# Autodesk Inventor assembly: LegAssemblyRightFront
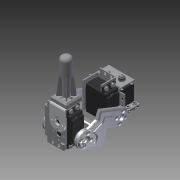
[picture p0: Inventor's stored thumbnail of the model, 180x180]
Saved by Autodesk Inventor 2015 (Build 190159000, 159)
## iProperties
Created: 2015-05-22
Part Number: LegAssemblyRightFront
Document SubType Name: Assembly
Designer: Quinn
Author: Quinn
## Documents named in this file (8)
- C:\Users\Quinn\Desktop\3DCNC Design\InventorModels\Assemblies\LegAssemblyRightFront.iam
- C:\Users\Quinn\Desktop\3DCNC Design\InventorModels\Assemblies\FXR_HipServo.iam
- C:\Users\Quinn\Desktop\3DCNC Design\InventorModels\Assemblies\LegAssemblyRightFront\Design Accelerator\Bolted Connection1.iam
- C:\Users\Quinn\Desktop\3DCNC Design\InventorModels\Assemblies\Knee_RightFront.iam
- C:\Users\Quinn\Desktop\3DCNC Design\InventorModels\Assemblies\FXL_HipServo.iam
- C:\Users\Quinn\Desktop\3DCNC Design\InventorModels\Assemblies\Foot.iam
- C:\Users\Quinn\Desktop\3DCNC Design\InventorModels\Assemblies\LegAssemblyRightFront\Design Accelerator\Bolted Connection2.iam
- C:\Users\Quinn\Desktop\3DCNC Design\InventorModels\Assemblies\LegAssemblyRightFront\Design Accelerator\Bolted Connection3.iam
## Components (8 placed, 5 different names)
1. FXR_HipServo:1 [sub-assembly] — Mate:1, Mate:2, Mate:3
2. FXR_HipServo:2 [sub-assembly] — Mate:1, Rotational:1
3. Bolted Connection:1 [sub-assembly] — Mate:2, Mate:3
4. Knee_RightFront:1 [sub-assembly] — Rotational:1, Rotational:2
5. FXL_HipServo:1 [sub-assembly] — Rotational:2, Mate:4, Mate:5, Mate:6
6. Foot:1 [sub-assembly] — Mate:4, Mate:5, Mate:6, Mate:7, Mate:8, Mate:9, Mate:10
7. Bolted Connection:2 [sub-assembly] — Mate:7, Mate:8
8. Bolted Connection:3 [sub-assembly] — Mate:9, Mate:10
## Relationships (12: Mate 10, RevoluteJoint 2)
- Mate:1: FXR_HipServo:1 ↔ FXR_HipServo:2
- Mate:2: FXR_HipServo:1 ↔ Bolted Connection:1
- Mate:3: FXR_HipServo:1 ↔ Bolted Connection:1
- Rotational:1 [RevoluteJoint]: FXR_HipServo:2 ↔ Knee_RightFront:1
- Rotational:2 [RevoluteJoint]: Knee_RightFront:1 ↔ FXL_HipServo:1
- Mate:4: FXL_HipServo:1 ↔ Foot:1
- Mate:5: FXL_HipServo:1 ↔ Foot:1
- Mate:6: FXL_HipServo:1 ↔ Foot:1
- Mate:7: Foot:1 ↔ Bolted Connection:2
- Mate:8: Foot:1 ↔ Bolted Connection:2
- Mate:9: Foot:1 ↔ Bolted Connection:3
- Mate:10: Foot:1 ↔ Bolted Connection:3
